# Autodesk Inventor assembly: GRINDING WHEEL
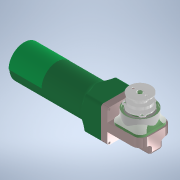
[picture p0: Inventor's stored thumbnail of the model, 180x180]
Saved by Autodesk Inventor 2020 (Build 240168000, 168)
## iProperties
Created: 2020-06-14
Part Number: GRINDING WHEEL
Document SubType Name: Assembly
Designer: Gebruiker
Author: Gebruiker
## Documents named in this file (9)
- C:\Users\Gebruiker\Documents\GitHub\BeerMinder\GRINDING WHEEL.iam
- C:\Users\Gebruiker\Documents\GitHub\DFA_THIJS\AS_1.ipt
- C:\Users\Gebruiker\Documents\GitHub\DFA_THIJS\GEAR_BOX.ipt
- C:\Users\Gebruiker\Documents\GitHub\DFA_THIJS\GEARPART.ipt
- C:\Users\Gebruiker\Documents\GitHub\DFA_THIJS\GRINDER_CASING.ipt
- C:\Users\Gebruiker\Documents\GitHub\DFA_THIJS\PART2.ipt
- C:\Users\Gebruiker\Documents\GitHub\DFA_THIJS\PART3.ipt
- C:\Users\Gebruiker\Documents\GitHub\DFA_THIJS\PART4.ipt
- C:\Users\Gebruiker\Documents\GitHub\DFA_THIJS\CASING_KLEP.ipt
## Components (9 placed, 8 different names)
1. AS_1:1 — Mate:1
2. GEAR_BOX:1 — Mate:1, Mate:2, Mate:3, Flush:1, Flush:2
3. GEARPART:1 — Mate:2, Mate:4, Mate:5, Mate:6
4. GRINDER_CASING:1 — Mate:3, Flush:1, Flush:2, Flush:3, Mate:7
5. PART2:1
6. PART2:2 — Mate:5
7. PART3:1 — Mate:4
8. PART4:1 — Mate:6
9. CASING_KLEP:1 — Flush:3, Mate:7
## Relationships (10: Mate 7, Flush 3)
- Mate:1: AS_1:1 ↔ GEAR_BOX:1
- Mate:2: GEAR_BOX:1 ↔ GEARPART:1
- Mate:3: GEAR_BOX:1 ↔ GRINDER_CASING:1
- Flush:1: GEAR_BOX:1 ↔ GRINDER_CASING:1
- Flush:2: GEAR_BOX:1 ↔ GRINDER_CASING:1
- Mate:4: GEARPART:1 ↔ PART3:1
- Mate:5: GEARPART:1 ↔ PART2:2
- Mate:6: GEARPART:1 ↔ PART4:1
- Flush:3: GRINDER_CASING:1 ↔ CASING_KLEP:1
- Mate:7: GRINDER_CASING:1 ↔ CASING_KLEP:1
